# Autodesk Inventor assembly: end door assembly (closed) (9).ipt
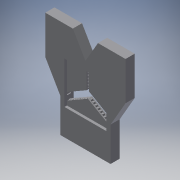
[picture p0: Inventor's stored thumbnail of the model, 180x180]
Saved by Autodesk Inventor 2017 (Build 210142000, 142)
## iProperties
Created: 2018-03-30
Part Number: end door assembly (closed) (9).ipt
Document SubType Name: Assembly
Designer: Braxton
Author: Braxton
## Documents named in this file (5)
- E:\School\Game develpment\geoscape\done\doors\end door\9 foot door\end door assembly (closed) (9).ipt.iam
- E:\School\Game develpment\geoscape\done\doors\end door\9 foot door\bottom door (9).ipt
- E:\School\Game develpment\geoscape\done\doors\end door\9 foot door\end door frame (9).ipt
- E:\School\Game develpment\geoscape\done\doors\end door\9 foot door\top left door (9).ipt
- E:\School\Game develpment\geoscape\done\doors\end door\9 foot door\top right door (9).ipt
## Components (4 placed, 4 different names)
1. end door frame (9):1 — Mate:2, Mate:6, Mate:7, Mate:8, Mate:9, Mate:10
2. bottom door (9):1 — Mate:2, Flush:2
3. top left door (9):1 — Mate:6, Mate:9, Flush:1, Mate:10, Flush:2, Flush:3
4. top right door (9):1 — Mate:7, Mate:8, Flush:1, Flush:3
## Relationships (9: Mate 6, Flush 3)
- Mate:2: end door frame (9):1 ↔ bottom door (9):1
- Mate:6: end door frame (9):1 ↔ top left door (9):1
- Mate:7: end door frame (9):1 ↔ top right door (9):1
- Mate:8: end door frame (9):1 ↔ top right door (9):1
- Mate:9: end door frame (9):1 ↔ top left door (9):1
- Flush:1: top left door (9):1 ↔ top right door (9):1
- Mate:10: end door frame (9):1 ↔ top left door (9):1
- Flush:2: bottom door (9):1 ↔ top left door (9):1
- Flush:3: top left door (9):1 ↔ top right door (9):1
